# Autodesk Inventor assembly: CAJA_P1
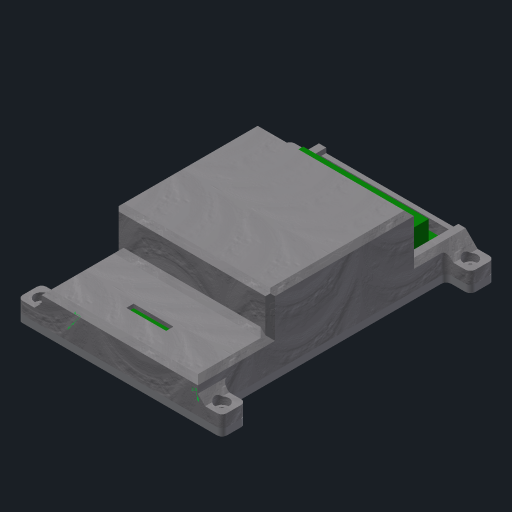
[picture p0: Inventor's stored thumbnail of the model, 512x512]
Saved by Autodesk Inventor 2024.3 (Build 283343000, 343)
## iProperties
Created: 2024-07-22
Part Number: CAJA_P1
Material: Generic
Document SubType Name: Assembly
Designer: Niler
Author: Niler
## Documents named in this file (4)
- C:\Users\Niler\OneDrive\Escritorio\RECICLADOR\RECICLADOR_MODELO_3D\DRIVER_MOTOR_DC\CAJA_P1.iam
- C:\Users\Niler\OneDrive\Escritorio\RECICLADOR\RECICLADOR_MODELO_3D\DRIVER_MOTOR_DC\DRIVER.ipt
- C:\Users\Niler\OneDrive\Escritorio\RECICLADOR\RECICLADOR_MODELO_3D\DRIVER_MOTOR_DC\CAJA_P1.ipt
- C:\Users\Niler\OneDrive\Escritorio\RECICLADOR\RECICLADOR_MODELO_3D\DRIVER_MOTOR_DC\CAJA_P2.ipt
## Components (3 placed, 3 different names)
1. DRIVER:1 — Flush:1, Mate:1, Flush:2
2. CAJA_P1:1 — Flush:1, Mate:1, Flush:2, Flush:3
3. CAJA_P2:1 — Flush:3
## Relationships (4: Flush 3, Mate 1)
- Flush:1 (2.5 mm): DRIVER:1 ↔ CAJA_P1:1
- Mate:1: DRIVER:1 ↔ CAJA_P1:1
- Flush:2: DRIVER:1 ↔ CAJA_P1:1
- Flush:3: CAJA_P1:1 ↔ CAJA_P2:1
